# Autodesk Inventor assembly: Ares v3_0
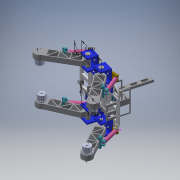
[picture p0: Inventor's stored thumbnail of the model, 180x180]
Saved by Autodesk Inventor 2018 (Build 220112000, 112)
## iProperties
Created: 2018-03-23
Part Number: Ares v3_0
Document SubType Name: Assembly
Designer: MIABo
Author: MIABo
## Documents named in this file (21)
- C:\Users\MIABo\Documents\GitHub\Ares1\3D Model Files\Ares v3_0.iam
- C:\Users\MIABo\Documents\GitHub\Ares1\3D Model Files\Frame 2.1.ipt
- C:\Users\MIABo\Documents\GitHub\Ares1\3D Model Files\Suspension Frame 3.0.ipt
- C:\Users\MIABo\Documents\GitHub\Ares1\3D Model Files\Frame mount rivet.ipt
- C:\Users\MIABo\Documents\GitHub\Ares1\3D Model Files\Leg Mount Rivet.ipt
- C:\Users\MIABo\Documents\GitHub\Ares1\3D Model Files\Leg Spacer.ipt
- C:\Users\MIABo\Documents\GitHub\Ares1\3D Model Files\Ares 2_0\Design Accelerator\Clevis Pin Connection1.iam
- C:\Users\MIABo\Documents\GitHub\Ares1\3D Model Files\Ares 2_0\Design Accelerator\Clevis Pin Connection2.iam
- C:\Users\MIABo\Documents\GitHub\Ares1\3D Model Files\Upper_Spring_Hanger.ipt
- C:\Users\MIABo\Documents\GitHub\Ares1\3D Model Files\leg 3.0.ipt
- C:\Users\MIABo\Documents\GitHub\Ares1\3D Model Files\SpringPin.ipt
- C:\Users\MIABo\Documents\GitHub\Ares1\3D Model Files\MockShock2.ipt
- C:\Users\MIABo\Documents\GitHub\Ares1\3D Model Files\LowerSpringMountRearBracket.ipt
- C:\Users\MIABo\Documents\GitHub\Ares1\3D Model Files\LowerSpringMountFront.ipt
- C:\Users\MIABo\Documents\GitHub\Ares1\3D Model Files\Upper_Spring_Hanger2.ipt
- C:\Users\MIABo\Documents\GitHub\Ares1\3D Model Files\wheel motor.ipt
- C:\Users\MIABo\Documents\GitHub\Ares1\3D Model Files\Rear Containment Thingy.ipt
- C:\Users\MIABo\Documents\GitHub\Ares1\3D Model Files\Pizza1.ipt
- C:\Users\MIABo\Documents\GitHub\Ares1\3D Model Files\Pizza2.ipt
- C:\Users\MIABo\Documents\GitHub\Ares1\3D Model Files\BatteryHanger.ipt
- C:\Users\MIABo\Documents\GitHub\Ares1\3D Model Files\arduino-mega-2560-rev3\Renderings\Autodesk Inventor Files\Assembly1.iam
## Components (72 placed, 19 different names)
1. Frame 2.1:1 — Mate:1, Mate:2, Mate:3, Mate:4, Mate:5, Mate:6, Mate:8, Mate:9, Mate:10, Mate:11, Mate:13, Mate:37, Flush:1, Mate:41, Mate:48, Mate:49
2. Suspension Frame 3.0:1 — Mate:1, Mate:2, Mate:4, Insert:5, Insert:6, Insert:9, Insert:16, Insert:22, Mate:31, Tangent:10, Tangent:11
3. Suspension Frame 3.0:2 — Mate:3, Mate:5, Mate:6, Insert:7, Insert:8, Insert:10, Insert:15, Insert:21, Mate:17, Insert:25, Insert:26
4. Suspension Frame 3.0:3 — Mate:8, Mate:9, Mate:10, Mate:12, Insert:2, Insert:3, Insert:11, Insert:13, Insert:20, Mate:16, Insert:29, Insert:30, Mate:43
5. Suspension Frame 3.0:4 — Mate:11, Mate:12, Mate:13, Insert:1, Insert:4, Insert:12, Insert:14, Mate:32, Tangent:13, Tangent:14
6. Frame mount rivet:1 — Insert:8
7. Frame mount rivet:2 — Insert:7
8. Frame mount rivet:3 — Insert:6
9. Frame mount rivet:4 — Insert:2
10. Frame mount rivet:5 — Insert:3
11. Frame mount rivet:6 — Insert:4
12. Frame mount rivet:7 — Insert:5
13. Frame mount rivet:8 — Insert:1
14. Leg Mount Rivet:1 — Insert:9
15. Leg Mount Rivet:2 — Insert:10
16. Leg Mount Rivet:3 — Insert:11
17. Leg Mount Rivet:4 — Insert:12
18. Leg Spacer:1 — Insert:22
19. Leg Spacer:2 — Insert:21
20. Leg Spacer:3 — Insert:20, Insert:33
21. Leg Spacer:4 — Insert:13
22. Leg Spacer:5 — Insert:14, Insert:34
23. Leg Spacer:6 — Insert:15, Insert:32
24. Leg Spacer:7 — Insert:16, Insert:31
25. Leg Spacer:8
26. Clevis Pin Connection:1 [sub-assembly]
27. Clevis Pin Connection:2 [sub-assembly]
28. Upper_Spring_Hanger:2 — Mate:16, Insert:29, Insert:30, Insert:37, Insert:38, Insert:57, Insert:58
29. Upper_Spring_Hanger:3 — Mate:17, Insert:25, Insert:26, Insert:45, Insert:46, Insert:61, Insert:62
30. leg 3.0:1 — Insert:31, Mate:27, Mate:28, Mate:29, Mate:36, Insert:56, Tangent:19
31. leg 3.0:2 — Insert:34, Mate:22, Mate:23, Mate:34, Insert:54, Tangent:17
32. leg 3.0:3 — Insert:33, Mate:19, Mate:20, Mate:35, Insert:53
33. leg 3.0:4 — Insert:32, Mate:25, Mate:26, Mate:30, Mate:33, Insert:55, Tangent:18
34. SpringPin:1 — Insert:38
35. SpringPin:2 — Insert:39, Mate:21
36. SpringPin:3 — Insert:49
37. SpringPin:4 — Insert:47, Tangent:8
38. SpringPin:5 — Insert:50
39. SpringPin:6 — Insert:45
40. SpringPin:7 — Insert:48, Tangent:15
41. SpringPin:8 — Insert:42, Tangent:16
42. MockShock2:1 — Insert:37, Mate:21
43. MockShock2:3 — Insert:46, Tangent:8
44. LowerSpringMountRearBracket:1 — Mate:27, Mate:28, Tangent:4, Tangent:5, Mate:36
45. LowerSpringMountRearBracket:2 — Mate:22, Mate:23, Mate:24, Tangent:1, Tangent:2, Mate:34
46. LowerSpringMountRearBracket:3 — Mate:25, Mate:26, Tangent:6, Tangent:7, Mate:33
47. LowerSpringMountRearBracket:4 — Mate:19, Mate:20, Insert:35, Insert:36, Mate:35
48. LowerSpringMountFront:1 — Mate:24, Tangent:1, Tangent:2, Insert:42
49. LowerSpringMountFront:2 — Insert:47, Mate:30, Tangent:6, Tangent:7
50. LowerSpringMountFront:3 — Insert:48, Mate:29, Tangent:4, Tangent:5
51. LowerSpringMountFront:4 — Insert:35, Insert:36, Insert:39
52. Upper_Spring_Hanger2:1 — Mate:32, Tangent:13, Tangent:14, Insert:50, Insert:52, Insert:59, Insert:60
53. Upper_Spring_Hanger2:2 — Mate:31, Tangent:10, Tangent:11, Insert:49, Insert:51, Insert:63, Insert:64
54. MockShock2:5 — Insert:52, Tangent:16
55. MockShock2:6 — Insert:51, Tangent:15
56. wheel motor:1 — Insert:53
57. wheel motor:2 — Insert:56, Tangent:19
58. wheel motor:3 — Insert:54, Tangent:17
59. wheel motor:4 — Insert:55, Tangent:18
60. Rear Containment Thingy:1 — Mate:41, Mate:42, Mate:43, Mate:44, Mate:46, Flush:2
61. Pizza1:1 — Mate:37, Flush:1, Mate:38, Mate:39, Mate:40, Mate:42
62. Pizza2:1 — Mate:38, Mate:39, Mate:40
63. BatteryHanger:1 — Mate:48, Mate:49
64. Assembly1:1 [sub-assembly] — Mate:44, Mate:46, Flush:2
65. Frame mount rivet:9 — Insert:63
66. Frame mount rivet:10 — Insert:64
67. Frame mount rivet:11 — Insert:60
68. Frame mount rivet:12 — Insert:62
69. Frame mount rivet:13 — Insert:61
70. Frame mount rivet:14 — Insert:59
71. Frame mount rivet:15 — Insert:58
72. Frame mount rivet:16 — Insert:57
## Relationships (114: Insert 53, Mate 43, Tangent 16, Flush 2)
- Mate:1: Frame 2.1:1 ↔ Suspension Frame 3.0:1
- Mate:2: Frame 2.1:1 ↔ Suspension Frame 3.0:1
- Mate:3: Frame 2.1:1 ↔ Suspension Frame 3.0:2
- Mate:4: Frame 2.1:1 ↔ Suspension Frame 3.0:1
- Mate:5: Frame 2.1:1 ↔ Suspension Frame 3.0:2
- Mate:6: Frame 2.1:1 ↔ Suspension Frame 3.0:2
- Mate:8: Frame 2.1:1 ↔ Suspension Frame 3.0:3
- Mate:9: Frame 2.1:1 ↔ Suspension Frame 3.0:3
- Mate:10: Frame 2.1:1 ↔ Suspension Frame 3.0:3
- Mate:11: Frame 2.1:1 ↔ Suspension Frame 3.0:4
- Mate:12: Suspension Frame 3.0:3 ↔ Suspension Frame 3.0:4
- Mate:13: Frame 2.1:1 ↔ Suspension Frame 3.0:4
- Insert:1 (-15.24 mm): Suspension Frame 3.0:4 ↔ Frame mount rivet:8
- Insert:2 (-15.24 mm): Suspension Frame 3.0:3 ↔ Frame mount rivet:4
- Insert:3 (-15.24 mm): Suspension Frame 3.0:3 ↔ Frame mount rivet:5
- Insert:4 (-15.24 mm): Suspension Frame 3.0:4 ↔ Frame mount rivet:6
- Insert:5 (-15.24 mm): Suspension Frame 3.0:1 ↔ Frame mount rivet:7
- Insert:6 (-15.24 mm): Suspension Frame 3.0:1 ↔ Frame mount rivet:3
- Insert:7 (-15.24 mm): Suspension Frame 3.0:2 ↔ Frame mount rivet:2
- Insert:8 (-15.24 mm): Suspension Frame 3.0:2 ↔ Frame mount rivet:1
- Insert:9: Suspension Frame 3.0:1 ↔ Leg Mount Rivet:1
- Insert:10: Suspension Frame 3.0:2 ↔ Leg Mount Rivet:2
- Insert:11: Suspension Frame 3.0:3 ↔ Leg Mount Rivet:3
- Insert:12: Suspension Frame 3.0:4 ↔ Leg Mount Rivet:4
- Insert:13: Suspension Frame 3.0:3 ↔ Leg Spacer:4
- Insert:14: Suspension Frame 3.0:4 ↔ Leg Spacer:5
- Insert:15: Suspension Frame 3.0:2 ↔ Leg Spacer:6
- Insert:16: Suspension Frame 3.0:1 ↔ Leg Spacer:7
- Insert:20: Suspension Frame 3.0:3 ↔ Leg Spacer:3
- Insert:21: Suspension Frame 3.0:2 ↔ Leg Spacer:2
- Insert:22: Suspension Frame 3.0:1 ↔ Leg Spacer:1
- Mate:16: Suspension Frame 3.0:3 ↔ Upper_Spring_Hanger:2
- Mate:17: Suspension Frame 3.0:2 ↔ Upper_Spring_Hanger:3
- Insert:25: Suspension Frame 3.0:2 ↔ Upper_Spring_Hanger:3
- Insert:26: Suspension Frame 3.0:2 ↔ Upper_Spring_Hanger:3
- Insert:29: Suspension Frame 3.0:3 ↔ Upper_Spring_Hanger:2
- Insert:30: Suspension Frame 3.0:3 ↔ Upper_Spring_Hanger:2
- Insert:31: Leg Spacer:7 ↔ leg 3.0:1
- Insert:32: Leg Spacer:6 ↔ leg 3.0:4
- Insert:33: Leg Spacer:3 ↔ leg 3.0:3
- Insert:34: Leg Spacer:5 ↔ leg 3.0:2
- Mate:19: leg 3.0:3 ↔ LowerSpringMountRearBracket:4
- Mate:20: leg 3.0:3 ↔ LowerSpringMountRearBracket:4
- Insert:35: LowerSpringMountRearBracket:4 ↔ LowerSpringMountFront:4
- Insert:36: LowerSpringMountRearBracket:4 ↔ LowerSpringMountFront:4
- Insert:37: Upper_Spring_Hanger:2 ↔ MockShock2:1
- Insert:38: Upper_Spring_Hanger:2 ↔ SpringPin:1
- Insert:39: SpringPin:2 ↔ LowerSpringMountFront:4
- Mate:21: SpringPin:2 ↔ MockShock2:1
- Mate:22: leg 3.0:2 ↔ LowerSpringMountRearBracket:2
- Mate:23: leg 3.0:2 ↔ LowerSpringMountRearBracket:2
- Mate:24: LowerSpringMountRearBracket:2 ↔ LowerSpringMountFront:1
- Tangent:1: LowerSpringMountRearBracket:2 ↔ LowerSpringMountFront:1
- Tangent:2: LowerSpringMountRearBracket:2 ↔ LowerSpringMountFront:1
- Insert:42: SpringPin:8 ↔ LowerSpringMountFront:1
- Insert:45: Upper_Spring_Hanger:3 ↔ SpringPin:6
- Insert:46: Upper_Spring_Hanger:3 ↔ MockShock2:3
- Mate:25: leg 3.0:4 ↔ LowerSpringMountRearBracket:3
- Mate:26: leg 3.0:4 ↔ LowerSpringMountRearBracket:3
- Mate:27: leg 3.0:1 ↔ LowerSpringMountRearBracket:1
- Mate:28: leg 3.0:1 ↔ LowerSpringMountRearBracket:1
- Insert:47: SpringPin:4 ↔ LowerSpringMountFront:2
- Insert:48: SpringPin:7 ↔ LowerSpringMountFront:3
- Mate:29: leg 3.0:1 ↔ LowerSpringMountFront:3
- Tangent:4: LowerSpringMountRearBracket:1 ↔ LowerSpringMountFront:3
- Tangent:5: LowerSpringMountRearBracket:1 ↔ LowerSpringMountFront:3
- Mate:30: leg 3.0:4 ↔ LowerSpringMountFront:2
- Tangent:6: LowerSpringMountRearBracket:3 ↔ LowerSpringMountFront:2
- Tangent:7: LowerSpringMountRearBracket:3 ↔ LowerSpringMountFront:2
- Tangent:8: SpringPin:4 ↔ MockShock2:3
- Mate:31: Suspension Frame 3.0:1 ↔ Upper_Spring_Hanger2:2
- Tangent:10: Suspension Frame 3.0:1 ↔ Upper_Spring_Hanger2:2
- Tangent:11: Suspension Frame 3.0:1 ↔ Upper_Spring_Hanger2:2
- Insert:49: SpringPin:3 ↔ Upper_Spring_Hanger2:2
- Mate:32: Suspension Frame 3.0:4 ↔ Upper_Spring_Hanger2:1
- Tangent:13: Suspension Frame 3.0:4 ↔ Upper_Spring_Hanger2:1
- Tangent:14: Suspension Frame 3.0:4 ↔ Upper_Spring_Hanger2:1
- Insert:50: SpringPin:5 ↔ Upper_Spring_Hanger2:1
- Insert:51: Upper_Spring_Hanger2:2 ↔ MockShock2:6
- Tangent:15: SpringPin:7 ↔ MockShock2:6
- Insert:52: Upper_Spring_Hanger2:1 ↔ MockShock2:5
- Tangent:16: SpringPin:8 ↔ MockShock2:5
- Mate:33: leg 3.0:4 ↔ LowerSpringMountRearBracket:3
- Mate:34: leg 3.0:2 ↔ LowerSpringMountRearBracket:2
- Mate:35: leg 3.0:3 ↔ LowerSpringMountRearBracket:4
- Mate:36: leg 3.0:1 ↔ LowerSpringMountRearBracket:1
- Mate:37: Frame 2.1:1 ↔ Pizza1:1
- Flush:1: Frame 2.1:1 ↔ Pizza1:1
- Mate:38: Pizza1:1 ↔ Pizza2:1
- Mate:39: Pizza1:1 ↔ Pizza2:1
- Mate:40: Pizza1:1 ↔ Pizza2:1
- Mate:41: Frame 2.1:1 ↔ Rear Containment Thingy:1
- Mate:42: Rear Containment Thingy:1 ↔ Pizza1:1
- Mate:43: Suspension Frame 3.0:3 ↔ Rear Containment Thingy:1
- Mate:44: Rear Containment Thingy:1 ↔ Assembly1:1
- Mate:46: Rear Containment Thingy:1 ↔ Assembly1:1
- Flush:2: Rear Containment Thingy:1 ↔ Assembly1:1
- Mate:48: Frame 2.1:1 ↔ BatteryHanger:1
- Mate:49: Frame 2.1:1 ↔ BatteryHanger:1
- Insert:53: leg 3.0:3 ↔ wheel motor:1
- Insert:54: leg 3.0:2 ↔ wheel motor:3
- Tangent:17: leg 3.0:2 ↔ wheel motor:3
- Insert:55: leg 3.0:4 ↔ wheel motor:4
- Tangent:18: leg 3.0:4 ↔ wheel motor:4
- Insert:56: leg 3.0:1 ↔ wheel motor:2
- Tangent:19: leg 3.0:1 ↔ wheel motor:2
- Insert:57: Upper_Spring_Hanger:2 ↔ Frame mount rivet:16
- Insert:58: Upper_Spring_Hanger:2 ↔ Frame mount rivet:15
- Insert:59: Upper_Spring_Hanger2:1 ↔ Frame mount rivet:14
- Insert:60: Upper_Spring_Hanger2:1 ↔ Frame mount rivet:11
- Insert:61: Upper_Spring_Hanger:3 ↔ Frame mount rivet:13
- Insert:62: Upper_Spring_Hanger:3 ↔ Frame mount rivet:12
- Insert:63: Upper_Spring_Hanger2:2 ↔ Frame mount rivet:9
- Insert:64: Upper_Spring_Hanger2:2 ↔ Frame mount rivet:10
